# Autodesk Inventor assembly: DriveChain2
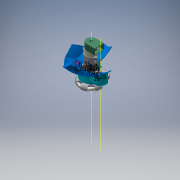
[picture p0: Inventor's stored thumbnail of the model, 180x180]
Saved by Autodesk Inventor 2018.3 (Build 223284000, 284)
## iProperties
Created: 2018-07-27
Part Number: DriveChain2
Material: Generisch
Document SubType Name: Assembly
Designer: JochenAlt
Author: JochenAlt
## Documents named in this file (14)
- D:\Projects\FlowerPot\CAD\DriveChain.iam
- D:\Projects\FlowerPot\CAD\Motor.iam
- D:\Projects\FlowerPot\CAD\HarmonicDrive-Axis.ipt
- D:\Projects\FlowerPot\CAD\BushOmniWheel.ipt
- D:\Projects\FlowerPot\CAD\OmniWheel-66mm.ipt
- D:\Projects\FlowerPot\CAD\Mounting Hub.ipt
- D:\Projects\FlowerPot\CAD\Encoder\Avago Encoder.iam
- D:\Projects\FlowerPot\CAD\DriveChainEnclosure2.ipt
- D:\Projects\FlowerPot\CAD\Spindle\SpindleThread.ipt
- D:\Projects\FlowerPot\CAD\Beltdrive\BeltDrive.iam
- D:\Projects\FlowerPot\CAD\AST_Bearings_SMR74ZZ.ipt
- C:\Users\JochenAlt\Documents\Inventor\Content Center Files\R2018\de-DE\SKF - Single row ball bearings\SKF623.ipt
- D:\Projects\FlowerPot\CAD\BeltDriveAxis.ipt
- D:\Projects\FlowerPot\CAD\BushBeltDriveTL.ipt
## Components (17 placed, 11 different names)
1. Motor:1 [sub-assembly] — Passend:44, Passend:53, Passend:58, Passend:59, Passend:60
2. HarmonicDrive-Axis:1 — Passend:11, Passend:13, Drehung:4, Passend:15, Fluchtend:1, Passend:71, Passend:82
3. BushOmniWheel:1 — Passend:11, Passend:14, Passend:73
4. OmniWheel:1 — Passend:15, Passend:16, Drehung:6, Fluchtend:1
5. Mounting Hub:1 — Passend:13, Drehung:4, Passend:14, Passend:16, Drehung:6
6. Avago Encoder:1 [sub-assembly] — Passend:57, Passend:58, Passend:59, Winkel:1
7. DriveChainEnclosure:1 — Passend:44, Passend:68, Passend:72, Passend:74, Passend:75, Passend:76, Passend:77, Passend:87, Passend:88
8. SpindleThread:1 — Passend:87, Passend:88
9. BeltDriveTest:1 [sub-assembly] — Passend:53, Passend:54, Passend:57, Passend:60, Passend:84, Passend:86
10. AST_Bearings_SMR74ZZ:1 — Passend:74, Passend:75, Passend:78, Fluchtend:2, Passend:81
11. AST_Bearings_SMR74ZZ:2 — Passend:76, Passend:77
12. SKF- Kugellager, einreihig SKF623:1 — Passend:68, Passend:71, Passend:72, Passend:73, Passend:83
13. HarmonicDrive-Axis:2 — Passend:78, Fluchtend:2, Passend:79, Passend:80, Passend:85
14. BushOmniWheel:2 — Passend:79
15. BushOmniWheel:3 — Passend:80, Passend:81
16. BushOmniWheel:4 — Passend:82, Passend:83, Passend:84
17. BushOmniWheel:5 — Passend:85, Passend:86
## Relationships (36: Mate 31, RelateRotation 2, Flush 2, Angle 1)
- Passend:11 [Mate]: HarmonicDrive-Axis:1 ↔ BushOmniWheel:1
- Passend:13 [Mate]: HarmonicDrive-Axis:1 ↔ Mounting Hub:1
- Drehung:4 [RelateRotation] (-1 ul): HarmonicDrive-Axis:1 ↔ Mounting Hub:1
- Passend:14 [Mate]: BushOmniWheel:1 ↔ Mounting Hub:1
- Passend:15 [Mate]: HarmonicDrive-Axis:1 ↔ OmniWheel:1
- Passend:16 [Mate]: OmniWheel:1 ↔ Mounting Hub:1
- Drehung:6 [RelateRotation] (1 ul): OmniWheel:1 ↔ Mounting Hub:1
- Passend:44 [Mate]: Motor:1 ↔ DriveChainEnclosure:1
- Passend:53 [Mate]: Motor:1 ↔ BeltDriveTest:1
- Passend:54 [Mate]: BeltDriveTest:1
- Passend:57 [Mate]: Avago Encoder:1 ↔ BeltDriveTest:1
- Passend:58 [Mate]: Motor:1 ↔ Avago Encoder:1
- Passend:59 [Mate] (0.5 mm): Motor:1 ↔ Avago Encoder:1
- Passend:60 [Mate] (0.5 mm): Motor:1 ↔ BeltDriveTest:1
- Passend:68 [Mate]: DriveChainEnclosure:1 ↔ SKF- Kugellager, einreihig SKF623:1
- Fluchtend:1 [Flush]: HarmonicDrive-Axis:1 ↔ OmniWheel:1
- Passend:71 [Mate]: HarmonicDrive-Axis:1 ↔ SKF- Kugellager, einreihig SKF623:1
- Passend:72 [Mate]: DriveChainEnclosure:1 ↔ SKF- Kugellager, einreihig SKF623:1
- Passend:73 [Mate]: BushOmniWheel:1 ↔ SKF- Kugellager, einreihig SKF623:1
- Passend:74 [Mate]: DriveChainEnclosure:1 ↔ AST_Bearings_SMR74ZZ:1
- Passend:75 [Mate]: DriveChainEnclosure:1 ↔ AST_Bearings_SMR74ZZ:1
- Passend:76 [Mate]: DriveChainEnclosure:1 ↔ AST_Bearings_SMR74ZZ:2
- Passend:77 [Mate]: DriveChainEnclosure:1 ↔ AST_Bearings_SMR74ZZ:2
- Passend:78 [Mate]: AST_Bearings_SMR74ZZ:1 ↔ HarmonicDrive-Axis:2
- Fluchtend:2 [Flush]: AST_Bearings_SMR74ZZ:1 ↔ HarmonicDrive-Axis:2
- Passend:79 [Mate]: HarmonicDrive-Axis:2 ↔ BushOmniWheel:2
- Passend:80 [Mate]: HarmonicDrive-Axis:2 ↔ BushOmniWheel:3
- Passend:81 [Mate]: AST_Bearings_SMR74ZZ:1 ↔ BushOmniWheel:3
- Passend:82 [Mate]: HarmonicDrive-Axis:1 ↔ BushOmniWheel:4
- Passend:83 [Mate]: SKF- Kugellager, einreihig SKF623:1 ↔ BushOmniWheel:4
- Passend:84 [Mate]: BeltDriveTest:1 ↔ BushOmniWheel:4
- Passend:85 [Mate]: HarmonicDrive-Axis:2 ↔ BushOmniWheel:5
- Passend:86 [Mate]: BeltDriveTest:1 ↔ BushOmniWheel:5
- Passend:87 [Mate]: DriveChainEnclosure:1 ↔ SpindleThread:1
- Passend:88 [Mate]: DriveChainEnclosure:1 ↔ SpindleThread:1
- Winkel:1 [Angle] (0 deg): Avago Encoder:1
